# Autodesk Inventor assembly: na4,5
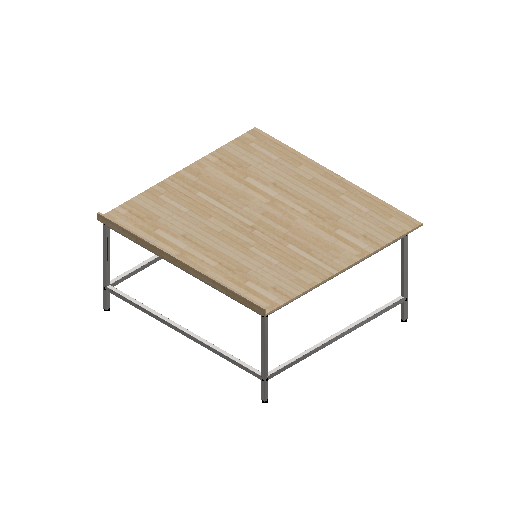
[picture p0: Inventor's stored thumbnail of the model, 512x512]
Saved by Autodesk Inventor 2025.1 (Build 291241000, 241)
## iProperties
Created: 2023-06-13
Part Number: na4,5
Document SubType Name: Assembly
Designer: MateuszWawrzyniak
_SolveAssemblyDoc: Frame Generator Solve Assembly
_Version: 25.0.0
Author: MateuszWawrzyniak
## Documents named in this file (4)
- C:\Users\Maciej\Desktop\Projekt_przej-ciowy\PP\modele\157339_Wawrzyniak\157339\na_4,5_157339\na4,5.iam
- C:\Users\Maciej\Desktop\Projekt_przej-ciowy\PP\modele\157339_Wawrzyniak\157339\na_4,5_157339\szkielet stolu.ipt
- C:\Users\Maciej\Desktop\Projekt_przej-ciowy\PP\modele\157339_Wawrzyniak\157339\na_4,5_157339\na4,5\Frame\Frame 1686649538613.iam
- C:\Users\Maciej\Desktop\Projekt_przej-ciowy\PP\modele\157339_Wawrzyniak\157339\na_4,5_157339\blat.ipt
## Components (3 placed, 3 different names)
1. szkielet stolu:1
2. Frame 1686649538613:1 [sub-assembly] — Zestawiające:1, Równoległe:1, Równoległe:2
3. blat:1 — Zestawiające:1, Równoległe:1, Równoległe:2
## Relationships (3: Flush 2, Mate 1)
- Zestawiające:1 [Mate]: Frame 1686649538613:1 ↔ blat:1
- Równoległe:1 [Flush] (-30 mm): Frame 1686649538613:1 ↔ blat:1
- Równoległe:2 [Flush] (-30 mm): Frame 1686649538613:1 ↔ blat:1
